# Autodesk Inventor assembly: Robot
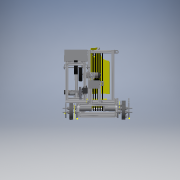
[picture p0: Inventor's stored thumbnail of the model, 180x180]
Saved by Autodesk Inventor 2016 (Build 200138000, 138)
## iProperties
Created: 2016-10-08
Part Number: Robot
Document SubType Name: Assembly
Designer: RoboticsUser
Author: RoboticsUser
## Documents named in this file (19)
- C:\Robotics\CAD\2016-17_CAD\Robot.iam
- C:\Robotics\CAD\2016-17_CAD\WheelAssemblyWFrame.iam
- C:\Robotics\CAD\COTSParts\Bosch Extrusion\Bosch 20x20 9 in.ipt
- C:\Robotics\CAD\COTSParts\Bosch Extrusion\Gusset 20x20 w screws.ipt
- C:\Robotics\CAD\COTSParts\Bosch Extrusion\Bosch 20x20 9 in - Copy.ipt
- C:\Robotics\CAD\COTSParts\Bosch Extrusion\Rexroth-6mmT-Nutm4.ipt
- C:\Robotics\CAD\COTSParts\Bosch Extrusion\Rexroth-GussetwFastenersm4x8.ipt
- C:\Robotics\CAD\COTSParts\Bosch Extrusion\Bosch 20x20 8.937in.ipt
- C:\Robotics\CAD\COTSParts\Bosch Extrusion\Bosch 20x20 9 in actual.ipt
- C:\Robotics\CAD\2016-17_CAD\ParticleLauncher2.0.iam
- C:\Robotics\CAD\2016-17_CAD\BBP.iam
- C:\Robotics\CAD\2016-17_CAD\ElectronicsPlate2.ipt
- C:\Robotics\CAD\2016-17_CAD\Deflecter.ipt
- C:\Robotics\CAD\COTSParts\Actobotics\585 parts\585424.ipt
- C:\Robotics\CAD\2016-17_CAD\14inLift - Copy.iam
- C:\Robotics\CAD\COTSParts\Bosch Extrusion\Bosch 20x20 4 14in.ipt
- C:\Robotics\CAD\2016-17_CAD\Backstop.iam
- C:\Robotics\CAD\COTSParts\Bosch Extrusion\Bosch 20x20 9 in actual2.ipt
- C:\Robotics\CAD\2016-17_CAD\CollectorPrototype.iam
## Components (42 placed, 18 different names)
1. WheelAssemblyWFrame:1 [sub-assembly] — Mate:1, Insert:4, Insert:5, Insert:6, Flush:29, Flush:37, Flush:42, Flush:114, Mate:181
2. WheelAssemblyWFrame:2 [sub-assembly] — Mate:8, Insert:1, Insert:2, Insert:3, Flush:30, Mate:57, Mate:58, Mate:77, Mate:192, Mate:194, Flush:122, Flush:123
3. Bosch 20x20 9 in:1 — Flush:37, Mate:56, Mate:58, Mate:69, Mate:70, Mate:71, Mate:72, Flush:42, Mate:73, Flush:43, Mate:75, Flush:44, Mate:77, Mate:180
4. Gusset 20x20 w screws:2 — Mate:1
5. Gusset 20x20 w screws:3 — Mate:8
6. Bosch 20x20 9 in - Copy:1 — Mate:33, Flush:25, Flush:28, Flush:30, Mate:44, Flush:34, Mate:175, Mate:183, Flush:115
7. Rexroth-6mmT-Nutm4:1 — Insert:1
8. Rexroth-6mmT-Nutm4:2 — Insert:3, Mate:33, Flush:25
9. Rexroth-6mmT-Nutm4:3 — Insert:2
10. Bosch 20x20 9 in - Copy:2 — Mate:15, Flush:11, Mate:39, Flush:29, Flush:32, Mate:48, Flush:33, Flush:116
11. Rexroth-6mmT-Nutm4:4 — Insert:4
12. Rexroth-6mmT-Nutm4:5 — Insert:5
13. Rexroth-6mmT-Nutm4:6 — Insert:6, Mate:15, Flush:11
14. Bosch 20x20 9 in:4 — Mate:39, Flush:28, Flush:32, Mate:45, Mate:46, Mate:47, Mate:49, Flush:33, Flush:34, Flush:111
15. Gusset 20x20 w screws:7 — Mate:47, Mate:48, Mate:49
16. Gusset 20x20 w screws:8 — Mate:44, Mate:45, Mate:46
17. Rexroth-GussetwFastenersm4x8:4 — Mate:56, Mate:57
18. Gusset 20x20 w screws:11 — Mate:70, Mate:71, Mate:76
19. Gusset 20x20 w screws:12 — Mate:69, Mate:72, Mate:74, Mate:182
20. Bosch 20x20 9 in actual:1 — Mate:73, Flush:43, Mate:74, Flush:66, Mate:104, Flush:68
21. Bosch 20x20 9 in actual:2 — Mate:75, Flush:44, Mate:76, Mate:100, Mate:101, Mate:102, Flush:67, Mate:126
22. Bosch 20x20 8.937in:4 — Mate:93, Flush:62, Flush:92, Flush:103, Flush:104, Mate:160
23. ParticleLauncher2.0:1 [sub-assembly] — Flush:103, Flush:104, Mate:160, Mate:163, Mate:164, Mate:165, Mate:166, Mate:168, Mate:169, Mate:170, Mate:171, Mate:174, Flush:113, Flush:114, Mate:180, Mate:181, Mate:182
24. Gusset 20x20 w screws:18 — Mate:93, Flush:62, Flush:92
25. BBP:1 [sub-assembly] — Mate:100, Mate:101, Flush:66, Mate:103, Mate:105, Mate:126
26. Gusset 20x20 w screws:21 — Mate:104, Mate:105, Flush:68
27. Gusset 20x20 w screws:22 — Mate:102, Mate:103, Flush:67
28. ElectronicsPlate2:1 — Mate:175, Flush:111
29. Deflecter:2 — Mate:174, Mate:177, Flush:112, Mate:179
30. 585424:2 — Insert:7, Insert:8, Flush:112, Mate:179, Flush:113
31. Rexroth-6mmT-Nutm4:7 — Mate:165, Mate:166, Insert:9
32. Rexroth-6mmT-Nutm4:8 — Mate:163, Mate:164, Insert:10
33. Rexroth-6mmT-Nutm4:10 — Mate:168, Mate:169, Insert:8
34. Rexroth-6mmT-Nutm4:11 — Mate:170, Mate:171, Insert:7
35. 585424:3 — Insert:9, Insert:10, Mate:177
36. 14inLift - Copy:1 [sub-assembly] — Mate:183, Flush:115, Flush:116, Mate:184, Flush:117, Mate:187, Mate:188, Flush:118, Mate:193, Flush:119, Flush:120, Flush:121
37. Bosch 20x20 4 14in:1 — Mate:184, Flush:117, Mate:185
38. Backstop:1 [sub-assembly] — Mate:185, Mate:190, Mate:191
39. Bosch 20x20 4 14in:2 — Mate:188, Flush:118, Mate:191, Flush:121
40. Bosch 20x20 4 14in:3 — Mate:187, Mate:190, Flush:120
41. Bosch 20x20 9 in actual2:1 — Mate:192, Mate:193, Flush:119
42. CollectorPrototype:1 [sub-assembly] — Mate:194, Flush:122, Flush:123
## Relationships (99: Mate 57, Flush 32, Insert 10)
- Mate:1: WheelAssemblyWFrame:1 ↔ Gusset 20x20 w screws:2
- Mate:8: WheelAssemblyWFrame:2 ↔ Gusset 20x20 w screws:3
- Insert:1: WheelAssemblyWFrame:2 ↔ Rexroth-6mmT-Nutm4:1
- Insert:2: WheelAssemblyWFrame:2 ↔ Rexroth-6mmT-Nutm4:3
- Insert:3: WheelAssemblyWFrame:2 ↔ Rexroth-6mmT-Nutm4:2
- Insert:4: WheelAssemblyWFrame:1 ↔ Rexroth-6mmT-Nutm4:4
- Insert:5: WheelAssemblyWFrame:1 ↔ Rexroth-6mmT-Nutm4:5
- Insert:6: WheelAssemblyWFrame:1 ↔ Rexroth-6mmT-Nutm4:6
- Mate:15: Bosch 20x20 9 in - Copy:2 ↔ Rexroth-6mmT-Nutm4:6
- Flush:11 (64.77 mm): Bosch 20x20 9 in - Copy:2 ↔ Rexroth-6mmT-Nutm4:6
- Mate:33: Bosch 20x20 9 in - Copy:1 ↔ Rexroth-6mmT-Nutm4:2
- Flush:25 (64.77 mm): Bosch 20x20 9 in - Copy:1 ↔ Rexroth-6mmT-Nutm4:2
- Mate:39: Bosch 20x20 9 in - Copy:2 ↔ Bosch 20x20 9 in:4
- Flush:28: Bosch 20x20 9 in - Copy:1 ↔ Bosch 20x20 9 in:4
- Flush:29 (1.6256 mm): WheelAssemblyWFrame:1 ↔ Bosch 20x20 9 in - Copy:2
- Flush:30 (1.6256 mm): WheelAssemblyWFrame:2 ↔ Bosch 20x20 9 in - Copy:1
- Flush:32: Bosch 20x20 9 in - Copy:2 ↔ Bosch 20x20 9 in:4
- Mate:44: Bosch 20x20 9 in - Copy:1 ↔ Gusset 20x20 w screws:8
- Mate:45: Bosch 20x20 9 in:4 ↔ Gusset 20x20 w screws:8
- Mate:46: Bosch 20x20 9 in:4 ↔ Gusset 20x20 w screws:8
- Mate:47: Bosch 20x20 9 in:4 ↔ Gusset 20x20 w screws:7
- Mate:48: Bosch 20x20 9 in - Copy:2 ↔ Gusset 20x20 w screws:7
- Mate:49: Bosch 20x20 9 in:4 ↔ Gusset 20x20 w screws:7
- Flush:33: Bosch 20x20 9 in - Copy:2 ↔ Bosch 20x20 9 in:4
- Flush:34: Bosch 20x20 9 in - Copy:1 ↔ Bosch 20x20 9 in:4
- Flush:37: WheelAssemblyWFrame:1 ↔ Bosch 20x20 9 in:1
- Mate:56: Bosch 20x20 9 in:1 ↔ Rexroth-GussetwFastenersm4x8:4
- Mate:57: WheelAssemblyWFrame:2 ↔ Rexroth-GussetwFastenersm4x8:4
- Mate:58: WheelAssemblyWFrame:2 ↔ Bosch 20x20 9 in:1
- Mate:69: Bosch 20x20 9 in:1 ↔ Gusset 20x20 w screws:12
- Mate:70: Bosch 20x20 9 in:1 ↔ Gusset 20x20 w screws:11
- Mate:71: Bosch 20x20 9 in:1 ↔ Gusset 20x20 w screws:11
- Mate:72: Bosch 20x20 9 in:1 ↔ Gusset 20x20 w screws:12
- Flush:42: WheelAssemblyWFrame:1 ↔ Bosch 20x20 9 in:1
- Mate:73: Bosch 20x20 9 in:1 ↔ Bosch 20x20 9 in actual:1
- Flush:43: Bosch 20x20 9 in:1 ↔ Bosch 20x20 9 in actual:1
- Mate:74: Gusset 20x20 w screws:12 ↔ Bosch 20x20 9 in actual:1
- Mate:75: Bosch 20x20 9 in:1 ↔ Bosch 20x20 9 in actual:2
- Flush:44: Bosch 20x20 9 in:1 ↔ Bosch 20x20 9 in actual:2
- Mate:76: Gusset 20x20 w screws:11 ↔ Bosch 20x20 9 in actual:2
- Mate:77: WheelAssemblyWFrame:2 ↔ Bosch 20x20 9 in:1
- Mate:93: Bosch 20x20 8.937in:4 ↔ Gusset 20x20 w screws:18
- Flush:62: Bosch 20x20 8.937in:4 ↔ Gusset 20x20 w screws:18
- Mate:100: Bosch 20x20 9 in actual:2 ↔ BBP:1
- Mate:101: Bosch 20x20 9 in actual:2 ↔ BBP:1
- Flush:66: Bosch 20x20 9 in actual:1 ↔ BBP:1
- Mate:102: Bosch 20x20 9 in actual:2 ↔ Gusset 20x20 w screws:22
- Mate:103: BBP:1 ↔ Gusset 20x20 w screws:22
- Flush:67: Bosch 20x20 9 in actual:2 ↔ Gusset 20x20 w screws:22
- Mate:104: Bosch 20x20 9 in actual:1 ↔ Gusset 20x20 w screws:21
- Mate:105: BBP:1 ↔ Gusset 20x20 w screws:21
- Flush:68: Bosch 20x20 9 in actual:1 ↔ Gusset 20x20 w screws:21
- Mate:126: Bosch 20x20 9 in actual:2 ↔ BBP:1
- Flush:92: Bosch 20x20 8.937in:4 ↔ Gusset 20x20 w screws:18
- Flush:103: Bosch 20x20 8.937in:4 ↔ ParticleLauncher2.0:1
- Flush:104: Bosch 20x20 8.937in:4 ↔ ParticleLauncher2.0:1
- Mate:160: Bosch 20x20 8.937in:4 ↔ ParticleLauncher2.0:1
- Mate:163: ParticleLauncher2.0:1 ↔ Rexroth-6mmT-Nutm4:8
- Mate:164: ParticleLauncher2.0:1 ↔ Rexroth-6mmT-Nutm4:8
- Mate:165: ParticleLauncher2.0:1 ↔ Rexroth-6mmT-Nutm4:7
- Mate:166: ParticleLauncher2.0:1 ↔ Rexroth-6mmT-Nutm4:7
- Mate:168: ParticleLauncher2.0:1 ↔ Rexroth-6mmT-Nutm4:10
- Mate:169: ParticleLauncher2.0:1 ↔ Rexroth-6mmT-Nutm4:10
- Mate:170: ParticleLauncher2.0:1 ↔ Rexroth-6mmT-Nutm4:11
- Mate:171: ParticleLauncher2.0:1 ↔ Rexroth-6mmT-Nutm4:11
- Mate:174: ParticleLauncher2.0:1 ↔ Deflecter:2
- Mate:175: Bosch 20x20 9 in - Copy:1 ↔ ElectronicsPlate2:1
- Flush:111 (7.3914 mm): Bosch 20x20 9 in:4 ↔ ElectronicsPlate2:1
- Insert:7: 585424:2 ↔ Rexroth-6mmT-Nutm4:11
- Insert:8: 585424:2 ↔ Rexroth-6mmT-Nutm4:10
- Insert:9: Rexroth-6mmT-Nutm4:7 ↔ 585424:3
- Insert:10: Rexroth-6mmT-Nutm4:8 ↔ 585424:3
- Mate:177: Deflecter:2 ↔ 585424:3
- Flush:112 (2.54 mm): Deflecter:2 ↔ 585424:2
- Mate:179: Deflecter:2 ↔ 585424:2
- Flush:113 (-88.9 mm): ParticleLauncher2.0:1 ↔ 585424:2
- Flush:114: WheelAssemblyWFrame:1 ↔ ParticleLauncher2.0:1
- Mate:180: Bosch 20x20 9 in:1 ↔ ParticleLauncher2.0:1
- Mate:181: WheelAssemblyWFrame:1 ↔ ParticleLauncher2.0:1
- Mate:182: Gusset 20x20 w screws:12 ↔ ParticleLauncher2.0:1
- Mate:183: Bosch 20x20 9 in - Copy:1 ↔ 14inLift - Copy:1
- Flush:115: Bosch 20x20 9 in - Copy:1 ↔ 14inLift - Copy:1
- Flush:116 (114.3 mm): Bosch 20x20 9 in - Copy:2 ↔ 14inLift - Copy:1
- Mate:184: 14inLift - Copy:1 ↔ Bosch 20x20 4 14in:1
- Flush:117: 14inLift - Copy:1 ↔ Bosch 20x20 4 14in:1
- Mate:185: Bosch 20x20 4 14in:1 ↔ Backstop:1
- Mate:187: 14inLift - Copy:1 ↔ Bosch 20x20 4 14in:3
- Mate:188: 14inLift - Copy:1 ↔ Bosch 20x20 4 14in:2
- Flush:118 (76.2 mm): 14inLift - Copy:1 ↔ Bosch 20x20 4 14in:2
- Mate:190: Backstop:1 ↔ Bosch 20x20 4 14in:3
- Mate:191: Backstop:1 ↔ Bosch 20x20 4 14in:2
- Mate:192: WheelAssemblyWFrame:2 ↔ Bosch 20x20 9 in actual2:1
- Mate:193: 14inLift - Copy:1 ↔ Bosch 20x20 9 in actual2:1
- Flush:119: 14inLift - Copy:1 ↔ Bosch 20x20 9 in actual2:1
- Flush:120: 14inLift - Copy:1 ↔ Bosch 20x20 4 14in:3
- Flush:121: 14inLift - Copy:1 ↔ Bosch 20x20 4 14in:2
- Mate:194: WheelAssemblyWFrame:2 ↔ CollectorPrototype:1
- Flush:122: WheelAssemblyWFrame:2 ↔ CollectorPrototype:1
- Flush:123 (25.4 mm): WheelAssemblyWFrame:2 ↔ CollectorPrototype:1
